# Autodesk Inventor assembly: Pneumatic_Compressor_VIAIR_00090
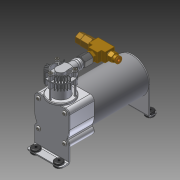
[picture p0: Inventor's stored thumbnail of the model, 180x180]
Saved by Autodesk Inventor 2014 SP1 (Build 180222100, 222)
## iProperties
Created: 2013-01-18
Part Number: Pneumatic_Compressor_VIAIR_00090
Document SubType Name: Assembly
Designer: Moses
Mass: 1088.62 g
Surface Area: 780.445 cm^2
Volume: 354.978 cm^3
Density: 3.06673 g/cm^3
Translation Standard: STEP AP214IS
FileName: E:\Data Folder\FIRST 2012\KOP\All Parts 2012\Pneumatics STEP\Pneumatic_Compressor_VIAIR_00090.stp
PreProcessor: Autodesk Inventor 2013
PostProcessor: Build: 138, Release: 2013 RTM - Date: Thu 03/01/2012
Sent Units: inch
Uncertainty: 0.00039370078740199997
Author: Moses
## Documents named in this file (15)
- C:\Users\Moses\Documents\Inventor\Sally Rebuild\Rebuild Sally\Pneumatic_Compressor_VIAIR_00090.iam
- C:\Users\Moses\Documents\Inventor\Sally Rebuild\Rebuild Sally\Pneumatics_VIAIR_0090_01.ipt
- C:\Users\Moses\Documents\Inventor\Sally Rebuild\Rebuild Sally\Pneumatics_VIAIR_0090_02.ipt
- C:\Users\Moses\Documents\Inventor\Sally Rebuild\Rebuild Sally\Pneumatics_VIAIR_00090_03.ipt
- C:\Users\Moses\Documents\Inventor\Sally Rebuild\Rebuild Sally\Pneumatics_VIAIR_0090_04.ipt
- C:\Users\Moses\Documents\Inventor\Sally Rebuild\Rebuild Sally\Pneumatic_VIAIR_Fitting.ipt
- C:\Users\Moses\Documents\Inventor\Sally Rebuild\Rebuild Sally\Pneumatics_VIAIR_Fitting_01.ipt
- C:\Users\Moses\Documents\Inventor\Sally Rebuild\Rebuild Sally\Pneumatics_VIAIR_00090_02.ipt
- C:\Users\Moses\Documents\Inventor\Sally Rebuild\Rebuild Sally\Hexagon Socket Head Cap Screw - Inch No. 5 - 40 UNC - 1 1_2.ipt
- C:\Users\Moses\Documents\Inventor\Sally Rebuild\Rebuild Sally\Hexagon Socket Button Head Cap Screw - Inch 6 - 32 x 1_4.ipt
- C:\Users\Moses\Documents\Inventor\Sally Rebuild\Rebuild Sally\Indented Large Hex Head Machine Screw - Inch 8-32 UNC - 1.25.ipt
- C:\Users\Moses\Documents\Inventor\Sally Rebuild\Rebuild Sally\Pneumatic_VIAIAR_00090_05.ipt
- C:\Users\Moses\Documents\Inventor\Sally Rebuild\Rebuild Sally\Pneumatics\Pneumatics_Parker_2203P-2.ipt
- C:\Users\Moses\Documents\Inventor\Sally Rebuild\Rebuild Sally\Pneumatics\Pneumatics_Parker_216P-2.ipt
- C:\Users\Moses\Documents\Inventor\Sally Rebuild\Rebuild Sally\Pneumatics\Pneumatics_SMC_KQ2H03-34S.ipt
## Components (24 placed, 14 different names)
1. Pneumatics_VIAIR_0090_01:1
2. Pneumatics_VIAIR_0090_02:1
3. Pneumatics_VIAIR_00090_03:1
4. Pneumatics_VIAIR_0090_04:1 — Insert:1, Insert:2, Insert:3
5. Pneumatic_VIAIR_Fitting:1 — Insert:6
6. Pneumatics_VIAIR_00090_02:1
7. Hexagon Socket Head Cap Screw - Inch No. 5 - 40 UNC - 1 1_2:1 — Insert:2
8. Hexagon Socket Head Cap Screw - Inch No. 5 - 40 UNC - 1 1_2:2 — Insert:1
9. Hexagon Socket Head Cap Screw - Inch No. 5 - 40 UNC - 1 1_2:3 — Insert:3
10. Hexagon Socket Button Head Cap Screw - Inch 6 - 32 x 1_4:1
11. Hexagon Socket Button Head Cap Screw - Inch 6 - 32 x 1_4:2
12. Hexagon Socket Button Head Cap Screw - Inch 6 - 32 x 1_4:3
13. Hexagon Socket Button Head Cap Screw - Inch 6 - 32 x 1_4:4
14. Indented Large Hex Head Machine Screw - Inch 8-32 UNC - 1.25:1
15. Indented Large Hex Head Machine Screw - Inch 8-32 UNC - 1.25:2
16. Pneumatic_VIAIAR_00090_05:1
17. Pneumatic_VIAIAR_00090_05:2
18. Pneumatic_VIAIAR_00090_05:3
19. Pneumatic_VIAIAR_00090_05:4
20. Pneumatic_VIAIR_Fitting:2 — Insert:4, Insert:8
21. Pneumatics_VIAIR_Fitting_01:2 — Insert:4
22. Pneumatics_Parker_2203P-2:1 — Insert:5, Insert:7, Insert:8
23. Pneumatics_Parker_216P-2:1 — Insert:5, Insert:6
24. Pneumatics_SMC_KQ2H03-34S:1 — Insert:7
## Relationships (8: Insert 8)
- Insert:1: Pneumatics_VIAIR_0090_04:1 ↔ Hexagon Socket Head Cap Screw - Inch No. 5 - 40 UNC - 1 1_2:2
- Insert:2: Pneumatics_VIAIR_0090_04:1 ↔ Hexagon Socket Head Cap Screw - Inch No. 5 - 40 UNC - 1 1_2:1
- Insert:3: Pneumatics_VIAIR_0090_04:1 ↔ Hexagon Socket Head Cap Screw - Inch No. 5 - 40 UNC - 1 1_2:3
- Insert:4 (0.508 mm): Pneumatic_VIAIR_Fitting:2 ↔ Pneumatics_VIAIR_Fitting_01:2
- Insert:5 (1.27 mm): Pneumatics_Parker_2203P-2:1 ↔ Pneumatics_Parker_216P-2:1
- Insert:6 (-5.08 mm): Pneumatic_VIAIR_Fitting:1 ↔ Pneumatics_Parker_216P-2:1
- Insert:7 (1.27 mm): Pneumatics_Parker_2203P-2:1 ↔ Pneumatics_SMC_KQ2H03-34S:1
- Insert:8 (1.27 mm): Pneumatic_VIAIR_Fitting:2 ↔ Pneumatics_Parker_2203P-2:1
